# Autodesk Inventor assembly: Samolot
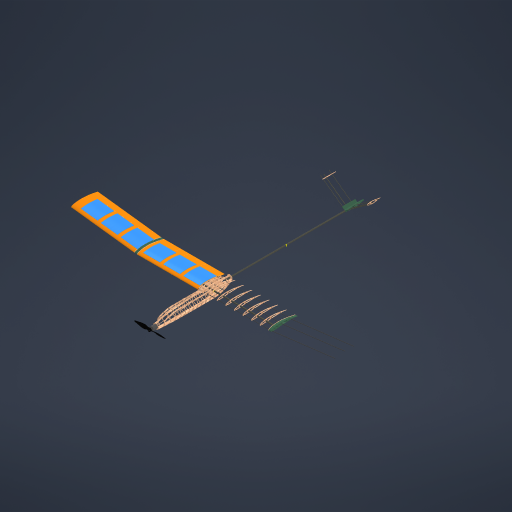
[picture p0: Inventor's stored thumbnail of the model, 512x512]
Saved by Autodesk Inventor 2023 (Build 270158000, 158)
## iProperties
Created: 2023-01-05
Part Number: Samolot
Document SubType Name: Assembly
Designer: szykr
Author: szykr
## Documents named in this file (12)
- D:\Folder Instalacyjny\GitHub Pliki\Solaris\new model\Samolot.iam
- D:\Folder Instalacyjny\GitHub Pliki\Solaris\new model\Skrzydło.iam
- D:\Folder Instalacyjny\GitHub Pliki\Solaris\new model\Tail\Tail.iam
- D:\Folder Instalacyjny\GitHub Pliki\Solaris\new model\nowy kadłub.ipt
- D:\Folder Instalacyjny\GitHub Pliki\Solaris\new model\Poszycie.ipt
- D:\Folder Instalacyjny\GitHub Pliki\Solaris\new model\Poszycie skrzydlo glowne.ipt
- D:\Folder Instalacyjny\GitHub Pliki\Solaris\new model\Poszycie skrzydlo sterowe.ipt
- D:\Folder Instalacyjny\GitHub Pliki\Solaris\new model\Silnik.ipt
- D:\Folder Instalacyjny\GitHub Pliki\Solaris\new model\APC_9x6.ipt
- D:\Folder Instalacyjny\GitHub Pliki\Solaris\new model\Panele.ipt
- D:\Folder Instalacyjny\GitHub Pliki\Solaris\new model\cienki_spar_dlugi.ipt
- D:\Folder Instalacyjny\GitHub Pliki\Solaris\new model\cienki_spar_krotki__ale_troche_dluzszy.ipt
## Components (35 placed, 11 different names)
1. Tail:1 [sub-assembly] — Insert:1
2. nowy kadłub:1 — Mate:1, Mate:2, Mate:3, Insert:1, Mate:4, Mate:5, Angle:1, Flush:6, Mate:17, Mate:19, Mate:21
3. Skrzydło:1 [sub-assembly] — Mate:1, Mate:2, Mate:3, Flush:1, Flush:2, Mate:6, Mate:7, Flush:3, Flush:4, Mate:8, Mate:9, Flush:5, Mate:10, Mate:11, Flush:8, Mate:12, Mate:13, Mate:14, Mate:15, Mate:16, Mate:18, Mate:20, Insert:3, Insert:4, Insert:5, Insert:6, Insert:7, Insert:8, Mate:23, Mate:24, Mate:26, Mate:27, Mate:29, Mate:30, Mate:32, Mate:33
4. Poszycie:1 — Mate:4, Mate:5, Angle:1
5. Poszycie skrzydlo glowne:1 — Flush:1, Flush:2
6. Poszycie skrzydlo glowne:2 — Mate:6, Mate:7, Flush:3, Flush:7
7. Poszycie skrzydlo sterowe:1 — Flush:4, Flush:9
8. Poszycie skrzydlo sterowe:2 — Mate:8, Mate:9, Flush:5, Flush:10
9. Silnik:1 — Flush:6, Insert:2
10. APC_9x6:1 — Insert:2
11. cienki_spar_dlugi:1 — Mate:16, Mate:17
12. cienki_spar_dlugi:2 — Mate:18, Mate:19
13. cienki_spar_dlugi:3 — Mate:20, Mate:21, Mate:28, Mate:31
14. cienki_spar_krotki__ale_troche_dluzszy:1 — Insert:3
15. cienki_spar_krotki__ale_troche_dluzszy:2 — Insert:4
16. cienki_spar_krotki__ale_troche_dluzszy:3 — Insert:5, Mate:22
17. cienki_spar_krotki__ale_troche_dluzszy:4 — Insert:8
18. cienki_spar_krotki__ale_troche_dluzszy:5 — Insert:7
19. cienki_spar_krotki__ale_troche_dluzszy:6 — Insert:6, Mate:25
20. Poszycie skrzydlo sterowe:3 — Mate:22, Mate:23, Mate:24
21. Poszycie skrzydlo sterowe:4 — Mate:25, Mate:26, Mate:27
22. Poszycie skrzydlo glowne:3 — Mate:28, Mate:29, Mate:30
23. Poszycie skrzydlo glowne:4 — Mate:31, Mate:32, Mate:33
24. Panele:1 — Flush:7
25. Panele:2
26. Panele:3
27. Panele:4 — Mate:10, Mate:11, Flush:8
28. Panele:5
29. Panele:6
30. Panele:7 — Mate:12, Mate:13, Flush:9
31. Panele:8
32. Panele:9
33. Panele:10 — Mate:14, Mate:15, Flush:10
34. Panele:11
35. Panele:12
## Component patterns: (3 elements, first: Panele:1), (3 elements, first: Panele:4), (3 elements, first: Panele:7), (3 elements, first: Panele:10)
## Relationships (52: Mate 33, Flush 10, Insert 8, Angle 1)
- Mate:1: nowy kadłub:1 ↔ Skrzydło:1
- Mate:2: nowy kadłub:1 ↔ Skrzydło:1
- Mate:3: nowy kadłub:1 ↔ Skrzydło:1
- Insert:1 (-40 mm): Tail:1 ↔ nowy kadłub:1
- Mate:4: nowy kadłub:1 ↔ Poszycie:1
- Mate:5: nowy kadłub:1 ↔ Poszycie:1
- Angle:1 (180 deg): nowy kadłub:1 ↔ Poszycie:1
- Flush:1: Skrzydło:1 ↔ Poszycie skrzydlo glowne:1
- Flush:2: Skrzydło:1 ↔ Poszycie skrzydlo glowne:1
- Mate:6: Skrzydło:1 ↔ Poszycie skrzydlo glowne:2
- Mate:7: Skrzydło:1 ↔ Poszycie skrzydlo glowne:2
- Flush:3: Skrzydło:1 ↔ Poszycie skrzydlo glowne:2
- Flush:4: Skrzydło:1 ↔ Poszycie skrzydlo sterowe:1
- Mate:8: Skrzydło:1 ↔ Poszycie skrzydlo sterowe:2
- Mate:9: Skrzydło:1 ↔ Poszycie skrzydlo sterowe:2
- Flush:5: Skrzydło:1 ↔ Poszycie skrzydlo sterowe:2
- Flush:6: nowy kadłub:1 ↔ Silnik:1
- Insert:2: Silnik:1 ↔ APC_9x6:1
- Flush:7: Poszycie skrzydlo glowne:2 ↔ Panele:1
- Mate:10: Skrzydło:1 ↔ Panele:4
- Mate:11: Skrzydło:1 ↔ Panele:4
- Flush:8: Skrzydło:1 ↔ Panele:4
- Mate:12: Skrzydło:1 ↔ Panele:7
- Mate:13: Skrzydło:1 ↔ Panele:7
- Flush:9: Poszycie skrzydlo sterowe:1 ↔ Panele:7
- Mate:14: Skrzydło:1 ↔ Panele:10
- Mate:15: Skrzydło:1 ↔ Panele:10
- Flush:10: Poszycie skrzydlo sterowe:2 ↔ Panele:10
- Mate:16: Skrzydło:1 ↔ cienki_spar_dlugi:1
- Mate:17: nowy kadłub:1 ↔ cienki_spar_dlugi:1
- Mate:18: Skrzydło:1 ↔ cienki_spar_dlugi:2
- Mate:19: nowy kadłub:1 ↔ cienki_spar_dlugi:2
- Mate:20: Skrzydło:1 ↔ cienki_spar_dlugi:3
- Mate:21: nowy kadłub:1 ↔ cienki_spar_dlugi:3
- Insert:3: Skrzydło:1 ↔ cienki_spar_krotki__ale_troche_dluzszy:1
- Insert:4: Skrzydło:1 ↔ cienki_spar_krotki__ale_troche_dluzszy:2
- Insert:5: Skrzydło:1 ↔ cienki_spar_krotki__ale_troche_dluzszy:3
- Insert:6: Skrzydło:1 ↔ cienki_spar_krotki__ale_troche_dluzszy:6
- Insert:7: Skrzydło:1 ↔ cienki_spar_krotki__ale_troche_dluzszy:5
- Insert:8: Skrzydło:1 ↔ cienki_spar_krotki__ale_troche_dluzszy:4
- Mate:22: cienki_spar_krotki__ale_troche_dluzszy:3 ↔ Poszycie skrzydlo sterowe:3
- Mate:23: Skrzydło:1 ↔ Poszycie skrzydlo sterowe:3
- Mate:24: Skrzydło:1 ↔ Poszycie skrzydlo sterowe:3
- Mate:25: cienki_spar_krotki__ale_troche_dluzszy:6 ↔ Poszycie skrzydlo sterowe:4
- Mate:26: Skrzydło:1 ↔ Poszycie skrzydlo sterowe:4
- Mate:27: Skrzydło:1 ↔ Poszycie skrzydlo sterowe:4
- Mate:28: cienki_spar_dlugi:3 ↔ Poszycie skrzydlo glowne:3
- Mate:29: Skrzydło:1 ↔ Poszycie skrzydlo glowne:3
- Mate:30: Skrzydło:1 ↔ Poszycie skrzydlo glowne:3
- Mate:31: cienki_spar_dlugi:3 ↔ Poszycie skrzydlo glowne:4
- Mate:32: Skrzydło:1 ↔ Poszycie skrzydlo glowne:4
- Mate:33: Skrzydło:1 ↔ Poszycie skrzydlo glowne:4
